# Autodesk Inventor assembly: CL4-300
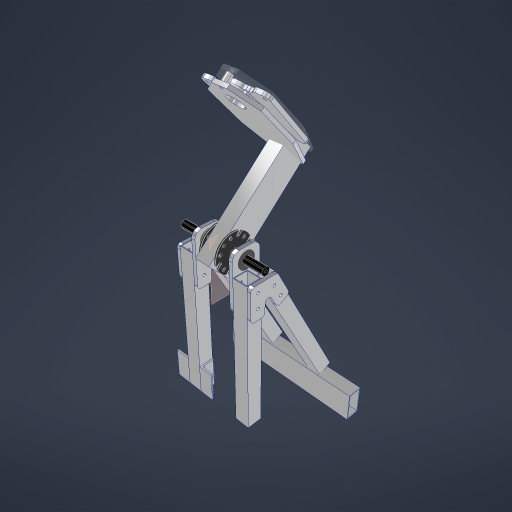
[picture p0: Inventor's stored thumbnail of the model, 512x512]
Saved by Autodesk Inventor 2023.4 (Build 274418000, 418)
## iProperties
Created: 2025-02-04
Part Number: CL4-300
Document SubType Name: Assembly
Designer: brand
Author: brand
## Documents named in this file (7)
- C:\Users\brand\OneDrive\Documents\GitHub\robotics 23\2025-ReefScape---CAD\Climber\CL4\CL4-300.iam
- C:\Users\brand\OneDrive\Documents\GitHub\robotics 23\2025-ReefScape---CAD\Climber\CL4\CL4-200.iam
- C:\Users\brand\OneDrive\Documents\GitHub\robotics 23\2025-ReefScape---CAD\Climber\CL4\CL4-100.iam
- C:\Users\brand\OneDrive\Documents\GitHub\robotics 23\2025-ReefScape---CAD\COMMON PARTS\BEARINGS\0_500_Hex_ID_x_1_125_OD_x_0_313_WD_Flanged_Bearing_v2_217-3875.ipt
- C:\Users\brand\OneDrive\Documents\GitHub\robotics 23\2025-ReefScape---CAD\Climber\CL4\CL4-011.ipt
- C:\Users\brand\OneDrive\Documents\GitHub\robotics 23\2025-ReefScape---CAD\Climber\CL4\CL4-012.ipt
- C:\Users\brand\OneDrive\Documents\GitHub\robotics 23\2025-ReefScape---CAD\Climber\CL4\CL4-013.ipt
## Components (8 placed, 6 different names)
1. CL4-200:1 [sub-assembly] — Insert:1, Insert:2, Angle:1, Flush:1, Mate:3, Mate:6, Mate:4, Flush:3, Flush:4, Mate:5, Flush:5, Flush:6
2. CL4-100:1 [sub-assembly] — Mate:2, Angle:1, Flush:1
3. 0_500_Hex_ID_x_1_125_OD_x_0_313_WD_Flanged_Bearing_v2_217-3875:1 — Insert:1, Mate:1
4. 0_500_Hex_ID_x_1_125_OD_x_0_313_WD_Flanged_Bearing_v2_217-3875:2 — Insert:2
5. CL4-011:1 — Mate:1, Mate:2
6. CL4-012:1 — Mate:3, Mate:6
7. CL4-013:1 — Mate:4, Flush:3, Flush:4
8. CL4-013:2 — Mate:5, Flush:5, Flush:6
## Relationships (14: Mate 6, Flush 5, Insert 2, Angle 1)
- Insert:1: CL4-200:1 ↔ 0_500_Hex_ID_x_1_125_OD_x_0_313_WD_Flanged_Bearing_v2_217-3875:1
- Insert:2: CL4-200:1 ↔ 0_500_Hex_ID_x_1_125_OD_x_0_313_WD_Flanged_Bearing_v2_217-3875:2
- Mate:1: 0_500_Hex_ID_x_1_125_OD_x_0_313_WD_Flanged_Bearing_v2_217-3875:1 ↔ CL4-011:1
- Mate:2: CL4-100:1 ↔ CL4-011:1
- Angle:1 (0 deg): CL4-200:1 ↔ CL4-100:1
- Flush:1: CL4-200:1 ↔ CL4-100:1
- Mate:3: CL4-200:1 ↔ CL4-012:1
- Mate:6: CL4-200:1 ↔ CL4-012:1
- Mate:4: CL4-200:1 ↔ CL4-013:1
- Flush:3: CL4-200:1 ↔ CL4-013:1
- Flush:4: CL4-200:1 ↔ CL4-013:1
- Mate:5: CL4-200:1 ↔ CL4-013:2
- Flush:5: CL4-200:1 ↔ CL4-013:2
- Flush:6: CL4-200:1 ↔ CL4-013:2
